# Autodesk Inventor assembly: DarkPoolFacility
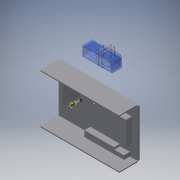
[picture p0: Inventor's stored thumbnail of the model, 180x180]
Saved by Autodesk Inventor 2019 (Build 230136000, 136)
## iProperties
Created: 2021-05-11
Part Number: DarkPoolFacility
Document SubType Name: Assembly
Designer: jamieson-bl
Author: jamieson-bl
## Documents named in this file (6)
- \\Mac\Home\Desktop\DarkPoolDrawings\DarkPoolFacility.iam
- \\Mac\Home\Desktop\DarkPoolDrawings\Room3L10.ipt
- \\Mac\Home\Desktop\DarkPoolDrawings\Pool.ipt
- \\Mac\Home\Desktop\DarkPoolDrawings\iManikins\iMan\iMan.iam
- \\Mac\Home\Desktop\DarkPoolDrawings\iManikins\iMandy\iMandy.iam
- \\Mac\Home\Desktop\DarkPoolDrawings\Field Compensation Coils.iam
## Components (5 placed, 5 different names)
1. Room3L10:1 — Mate:2, Mate:3
2. Pool:1 — Mate:4
3. iMan:1 [sub-assembly] — Mate:3
4. iMandy:1 [sub-assembly] — Mate:2
5. Field Compensation Coils:1 [sub-assembly] — Mate:4
## Relationships (3: Mate 3)
- Mate:2: Room3L10:1 ↔ iMandy:1
- Mate:3: Room3L10:1 ↔ iMan:1
- Mate:4: Pool:1 ↔ Field Compensation Coils:1
